# Autodesk Inventor assembly: LearningKitWater
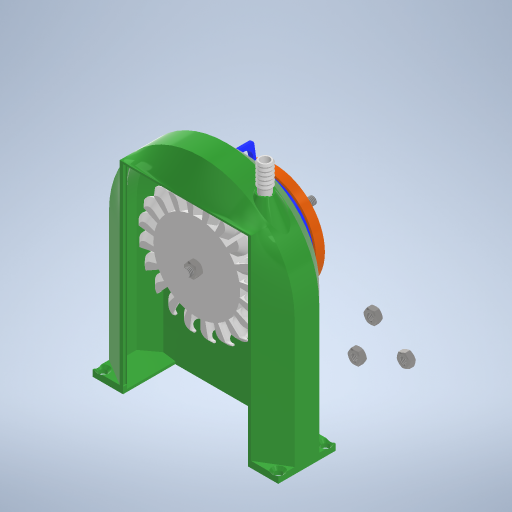
[picture p0: Inventor's stored thumbnail of the model, 512x512]
Saved by Autodesk Inventor 2024.3 (Build 283343000, 343)
## iProperties
Created: 2024-12-10
Part Number: LearningKitWater
Document SubType Name: Assembly
Designer: Maximilian Hock
Author: Maximilian Hock
## Documents named in this file (6)
- Z:\Dokumente\LearningKit\LearningKitWater\LearningKitWater.iam
- Z:\Dokumente\LearningKit\LearningKitWater\PeltonTurbine.ipt
- Z:\Dokumente\LearningKit\LearningKitGenerator\PancakeGenerator.iam
- Z:\Dokumente\LearningKit\LearningKitWater\TurbineHousingAlt.ipt
- Z:\Dokumente\LearningKit\LearningKitWater\TurbineNozzle.ipt
- Z:\Dokumente\Inventor\Content Center Files\R2024\de-DE\DIN EN ISO 4032\DIN EN ISO 4032 - M6.ipt
## Components (10 placed, 5 different names)
1. PeltonTurbine:1 — Zylindrisch:3
2. PancakeGenerator:1 [sub-assembly] — Zylindrisch:3, Zylindrisch:7, Planar:4
3. TurbineHousingAlt:1 — Fluchtend:2, Zylindrisch:7, Planar:4, Passend:1, Passend:2, Zylindrisch:8
4. DIN EN ISO 4032 M6:1
5. DIN EN ISO 4032 M6:2
6. DIN EN ISO 4032 M6:3
7. DIN EN ISO 4032 M6:4
8. DIN EN ISO 4032 M6:5
9. DIN EN ISO 4032 M6:6
10. TurbineNozzle:1 — Zylindrisch:8
## Relationships (14: CylindricalJoint 6, PlanarJoint 3, RevoluteJoint 2, Mate 2, Flush 1)
- Zylindrisch:3 [CylindricalJoint]: PeltonTurbine:1 ↔ PancakeGenerator:1
- [CylindricalJoint]: PancakeGenerator:1 ↔ DIN EN ISO 4032 M6:5
- [PlanarJoint]: PeltonTurbine:1 ↔ DIN EN ISO 4032 M6:5
- [CylindricalJoint]: PancakeGenerator:1 ↔ DIN EN ISO 4032 M6:4
- [PlanarJoint]: PeltonTurbine:1 ↔ DIN EN ISO 4032 M6:4
- [CylindricalJoint]: PancakeGenerator:1 ↔ DIN EN ISO 4032 M6:6
- [RevoluteJoint]: PancakeGenerator:1 ↔ DIN EN ISO 4032 M6:6
- [RevoluteJoint]: DIN EN ISO 4032 M6:5 ↔ DIN EN ISO 4032 M6:6
- Fluchtend:2 [Flush]: TurbineHousingAlt:1
- Zylindrisch:7 [CylindricalJoint]: PancakeGenerator:1 ↔ TurbineHousingAlt:1
- Planar:4: PancakeGenerator:1 ↔ TurbineHousingAlt:1
- Passend:1 [Mate]: TurbineHousingAlt:1
- Passend:2 [Mate]: TurbineHousingAlt:1
- Zylindrisch:8 [CylindricalJoint]: TurbineHousingAlt:1 ↔ TurbineNozzle:1
